# Autodesk Inventor assembly: PP
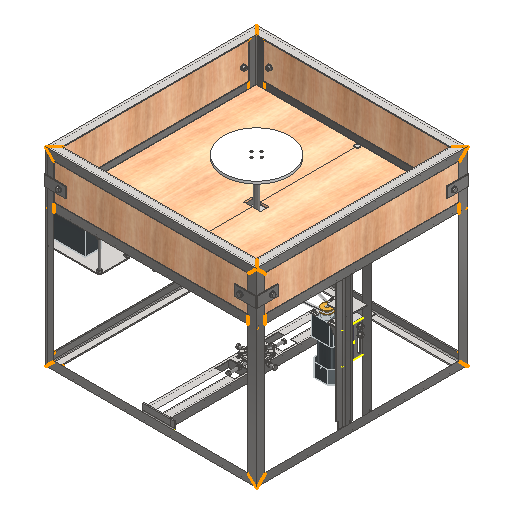
[picture p0: Inventor's stored thumbnail of the model, 512x512]
Saved by Autodesk Inventor 2025 (Build 290162000, 162)
## iProperties
Created: 2025-02-12
Part Number: PP
Document SubType Name: Weldment
Designer: teiko
Weld Material: Steel, Mild, Welded
Mass: 4.42779e+07 g
Surface Area: 1.45033e+06 cm^2
Volume: 5.65311e+06 cm^3
Density: 7.83248 g/cm^3
Author: teiko
## Documents named in this file (22)
- C:\Users\teiko\OneDrive\Documents\Inventor\Projectpotterpro\parts\PP.iam
- C:\Users\teiko\OneDrive\Documents\Inventor\Projectpotterpro\assembly\PP0101.iam
- C:\Users\teiko\OneDrive\Documents\Inventor\Projectpotterpro\parts\PP0306.iam
- C:\Users\teiko\OneDrive\Documents\Inventor\Content Center Files\R2025\en-US\ISO 7091\ISO 7091 - ST 12 - 100 HV.ipt
- C:\Users\teiko\OneDrive\Documents\Inventor\Content Center Files\R2025\en-US\ISO 4017(1)\ISO 4017 - M12 x 25 - ISO.ipt
- C:\Users\teiko\OneDrive\Documents\Inventor\Content Center Files\R2025\en-US\ISO 4032(2)\ISO 4032 - M12 - ISO.ipt
- C:\Users\teiko\OneDrive\Documents\Inventor\Projectpotterpro\parts\PP0501.ipt
- C:\Users\teiko\OneDrive\Documents\Inventor\Projectpotterpro\parts\PP0502.ipt
- C:\Users\teiko\OneDrive\Documents\Inventor\Projectpotterpro\parts\ISO 657-1 - L40x40x3-647.ipt
- C:\Users\teiko\OneDrive\Documents\Inventor\Projectpotterpro\parts\PP0411.iam
- C:\Users\teiko\OneDrive\Documents\Inventor\Projectpotterpro\parts\PP0412.ipt
- C:\Users\teiko\OneDrive\Documents\Inventor\Projectpotterpro\parts\PP0204.iam
- C:\Users\teiko\OneDrive\Documents\Inventor\Projectpotterpro\parts\6245K16_Pulley\6245K16_Pulley.ipt
- C:\Users\teiko\OneDrive\Documents\Inventor\Projectpotterpro\parts\PP0503.ipt
- C:\Users\teiko\OneDrive\Documents\Inventor\Content Center Files\R2025\en-US\ISO 4017(1)\ISO 4017 - M12 x 30 - ISO.ipt
- C:\Users\teiko\OneDrive\Documents\Inventor\Projectpotterpro\parts\PP0505.ipt
- C:\Users\teiko\OneDrive\Documents\Inventor\Projectpotterpro\parts\6245K541_Pulley\6245K541_Pulley.ipt
- C:\Users\teiko\OneDrive\Documents\Inventor\Projectpotterpro\parts\PP0504.ipt
- C:\Users\teiko\OneDrive\Documents\Inventor\Projectpotterpro\parts\PP\Design Accelerator\V-Belt transmission2.iam
- C:\Users\teiko\OneDrive\Documents\Inventor\Projectpotterpro\parts\PP0507.iam
- C:\Users\teiko\OneDrive\Documents\Inventor\Projectpotterpro\parts\PP0509.ipt
- C:\Users\teiko\OneDrive\Documents\Inventor\Projectpotterpro\parts\PP0510.ipt
## Components (79 placed, 21 different names)
1. PP0101:1 [sub-assembly] — Flush:1, Flush:2, Mate:1, Mate:5, Mate:6, Mate:7, Mate:9, Mate:10, Mate:11, Flush:10, Mate:31, Flush:18, Flush:19, Flush:22, Mate:51, Mate:73, Mate:74, Mate:81, Symmetry:2, Mate:92, Mate:93, Mate:106, Flush:97, Symmetry:3, Mate:107, Flush:98, Mate:109, Flush:100, Mate:115, Flush:104, Mate:125, Flush:108, Mate:130, Flush:109, Mate:131, Flush:111, Mate:132, Flush:114, Mate:133, Flush:116, Mate:134, Flush:118, Mate:135, Flush:120, Flush:122, Flush:123, Mate:154, Mate:155, Mate:163, Mate:164, Mate:165, Mate:170, Mate:172, Mate:178, Mate:180
2. ISO 7091 ST 12 - 100 HV:1 — Mate:5, Mate:6, Insert:1
3. ISO 4017 M12 x 25:1 — Insert:1, Mate:153
4. ISO 7091 ST 12 - 100 HV:2 — Mate:7, Insert:2
5. ISO 4032 M12:1 — Insert:2
6. ISO 7091 ST 12 - 100 HV:3 — Mate:9, Mate:10, Insert:3
7. ISO 4017 M12 x 25:2 — Insert:3, Mate:77, Mate:152
8. ISO 7091 ST 12 - 100 HV:4 — Mate:11, Mate:78
9. ISO 4032 M12:2 — Mate:77, Mate:78
10. PP0501:2 — Mate:92, Mate:93, Mate:114, Mate:119
11. PP0501:4 — Mate:107, Flush:98, Mate:108, Mate:124, Mate:129
12. PP0502:1 — Mate:31, Flush:18, Flush:19, Mate:52, Mate:53, Mate:83, Symmetry:3
13. PP0502:2 — Mate:51, Mate:52, Mate:53, Symmetry:2
14. ISO 657-1 - L40x40x3-647:1 — Mate:73, Mate:74, Mate:75, Flush:66, Symmetry:1
15. ISO 657-1 - L40x40x3-647:2 — Flush:66, Mate:81, Flush:67, Mate:82, Symmetry:1
16. PP0411:1 [sub-assembly] — Mate:82, Mate:83, Flush:68, Mate:84, Mate:96, Flush:124
17. PP0412:1 — Flush:69, Flush:70, Mate:85, Angle:1
18. ISO 4032 M12:3 — Mate:84, Mate:85, Angle:1
19. 6245K16_Pulley:1 — Mate:96, Flush:124, Flush:128
20. PP0503:1 — Mate:132, Flush:113, Flush:114, Flush:115, Mate:136, Mate:137, Mate:138
21. PP0503:2 — Mate:133, Flush:115, Flush:116, Flush:117, Mate:140, Mate:141, Mate:142
22. PP0503:3 — Mate:106, Flush:97, Mate:111, Mate:112, Mate:113, Flush:103, Flush:107
23. PP0503:4 — Mate:135, Flush:119, Flush:120, Mate:148, Mate:149, Mate:150
24. PP0503:7 — Mate:115, Flush:103, Flush:104, Mate:116, Mate:117, Mate:118, Flush:113, Flush:122
25. PP0503:8 — Mate:134, Flush:117, Flush:118, Mate:144, Mate:145, Mate:146
26. PP0503:9 — Mate:125, Flush:107, Flush:108, Mate:126, Mate:127, Mate:128
27. PP0503:10 — Mate:109, Flush:100, Mate:121, Mate:122, Mate:123, Flush:119, Flush:123
28. ISO 7091 ST 12 - 100 HV:5 — Mate:111, Mate:112, Insert:4
29. ISO 4017 M12 x 30:1 — Insert:4
30. ISO 7091 ST 12 - 100 HV:6 — Mate:113, Mate:114, Insert:5
31. ISO 4032 M12:4 — Insert:5
32. ISO 7091 ST 12 - 100 HV:7 — Mate:116, Mate:117, Insert:6
33. ISO 4017 M12 x 30:2 — Insert:6
34. ISO 7091 ST 12 - 100 HV:8 — Mate:118, Mate:119, Insert:7
35. ISO 4032 M12:5 — Insert:7
36. ISO 7091 ST 12 - 100 HV:9 — Mate:121, Mate:122, Insert:8
37. ISO 4017 M12 x 30:3 — Insert:8
38. ISO 7091 ST 12 - 100 HV:10 — Mate:123, Mate:124, Insert:9
39. ISO 4032 M12:6 — Insert:9
40. ISO 7091 ST 12 - 100 HV:11 — Mate:126, Mate:127, Insert:10
41. ISO 4017 M12 x 30:4 — Insert:10
42. ISO 7091 ST 12 - 100 HV:12 — Mate:128, Mate:129, Insert:11
43. ISO 4032 M12:7 — Insert:11
44. PP0505:1 — Mate:131, Flush:111, Flush:112, Mate:147, Mate:151
45. PP0505:2 — Mate:130, Flush:109, Flush:110, Mate:139, Mate:143
46. ISO 7091 ST 12 - 100 HV:13 — Mate:136, Mate:137, Insert:12
47. ISO 4017 M12 x 30:5 — Insert:12
48. ISO 7091 ST 12 - 100 HV:14 — Mate:138, Mate:139, Insert:13
49. ISO 4032 M12:8 — Insert:13
50. ISO 7091 ST 12 - 100 HV:15 — Mate:140, Mate:141, Insert:14
51. ISO 4017 M12 x 30:6 — Insert:14
52. ISO 7091 ST 12 - 100 HV:16 — Mate:142, Mate:143, Insert:15
53. ISO 4032 M12:9 — Insert:15
54. ISO 7091 ST 12 - 100 HV:17 — Mate:144, Mate:145, Insert:16
55. ISO 4017 M12 x 30:7 — Insert:16
56. ISO 7091 ST 12 - 100 HV:18 — Mate:146, Mate:147, Insert:17
57. ISO 4032 M12:10 — Insert:17
58. ISO 7091 ST 12 - 100 HV:19 — Mate:148, Mate:149, Insert:18
59. ISO 4017 M12 x 30:8 — Insert:18
60. ISO 7091 ST 12 - 100 HV:20 — Mate:150, Mate:151, Insert:19
61. ISO 4032 M12:11 — Insert:19
62. PP0306:1 [sub-assembly] — Mate:152, Mate:153, Mate:154, Flush:125, Flush:126
63. PP0306:2 [sub-assembly] — Flush:125, Flush:126, Mate:155, Mate:156, Flush:127
64. PP0204:1 [sub-assembly] — Mate:156, Flush:127, Mate:157, Mate:158, Mate:159, Mate:160, Mate:161
65. 6245K541_Pulley:1 — Mate:157, Flush:128, Mate:158
66. PP0504:1 — Mate:159, Mate:160, Mate:161
67. V-Belt transmission:1 [sub-assembly]
68. PP0507:1 [sub-assembly] — Mate:166, Mate:167, Mate:168, Flush:129
69. PP0509:1 — Mate:163, Mate:164, Mate:165, Insert:20, Insert:21, Insert:22, Insert:23, Mate:166, Mate:167, Mate:168, Flush:129, Mate:174, Mate:176
70. ISO 4032 M12:12 — Insert:20, Mate:169, Mate:175
71. ISO 4032 M12:13 — Insert:21, Mate:171, Mate:173
72. ISO 4032 M12:14 — Insert:22, Mate:177, Mate:179
73. ISO 4032 M12:15 — Insert:23
74. ISO 4032 M12:16 — Mate:169, Mate:170
75. ISO 4032 M12:17 — Mate:171, Mate:172
76. PP0510:1 — Mate:173, Mate:174
77. PP0510:2 — Mate:175, Mate:176
78. PP0510:3 — Mate:179, Mate:180
79. ISO 4032 M12:18 — Mate:177, Mate:178
## Relationships (162: Mate 96, Flush 39, Insert 23, Symmetry 3, Angle 1)
- Flush:1: PP0101:1
- Flush:2: PP0101:1
- Mate:1: PP0101:1
- Mate:5: PP0101:1 ↔ ISO 7091 ST 12 - 100 HV:1
- Mate:6: PP0101:1 ↔ ISO 7091 ST 12 - 100 HV:1
- Insert:1: ISO 7091 ST 12 - 100 HV:1 ↔ ISO 4017 M12 x 25:1
- Mate:7: PP0101:1 ↔ ISO 7091 ST 12 - 100 HV:2
- Insert:2: ISO 7091 ST 12 - 100 HV:2 ↔ ISO 4032 M12:1
- Mate:9: PP0101:1 ↔ ISO 7091 ST 12 - 100 HV:3
- Mate:10: PP0101:1 ↔ ISO 7091 ST 12 - 100 HV:3
- Insert:3: ISO 7091 ST 12 - 100 HV:3 ↔ ISO 4017 M12 x 25:2
- Mate:11: PP0101:1 ↔ ISO 7091 ST 12 - 100 HV:4
- Flush:10 (648.895 mm): PP0101:1
- Flush:12
- Mate:31: PP0101:1 ↔ PP0502:1
- Flush:18: PP0101:1 ↔ PP0502:1
- Flush:19: PP0101:1 ↔ PP0502:1
- Flush:22 (426.446 mm): PP0101:1
- Mate:51: PP0101:1 ↔ PP0502:2
- Mate:52: PP0502:1 ↔ PP0502:2
- Mate:53: PP0502:1 ↔ PP0502:2
- Mate:73: PP0101:1 ↔ ISO 657-1 - L40x40x3-647:1
- Mate:74 (-40 mm): PP0101:1 ↔ ISO 657-1 - L40x40x3-647:1
- Mate:75 (45 mm): ISO 657-1 - L40x40x3-647:1
- Mate:77: ISO 4017 M12 x 25:2 ↔ ISO 4032 M12:2
- Mate:78: ISO 7091 ST 12 - 100 HV:4 ↔ ISO 4032 M12:2
- Flush:66: ISO 657-1 - L40x40x3-647:1 ↔ ISO 657-1 - L40x40x3-647:2
- Mate:81: PP0101:1 ↔ ISO 657-1 - L40x40x3-647:2
- Flush:67 (-45 mm): ISO 657-1 - L40x40x3-647:2
- Mate:82: ISO 657-1 - L40x40x3-647:2 ↔ PP0411:1
- Symmetry:1: ISO 657-1 - L40x40x3-647:1 ↔ ISO 657-1 - L40x40x3-647:2
- Mate:83 (250 mm): PP0502:1 ↔ PP0411:1
- Flush:68 (60 mm): PP0411:1
- Flush:69: PP0412:1
- Flush:70: PP0412:1
- Mate:84: PP0411:1 ↔ ISO 4032 M12:3
- Mate:85: PP0412:1 ↔ ISO 4032 M12:3
- Angle:1 (0 deg): PP0412:1 ↔ ISO 4032 M12:3
- Symmetry:2: PP0101:1 ↔ PP0502:2
- Mate:92: PP0101:1 ↔ PP0501:2
- Mate:93: PP0101:1 ↔ PP0501:2
- Mate:96: PP0411:1 ↔ 6245K16_Pulley:1
- Mate:106: PP0101:1 ↔ PP0503:3
- Flush:97: PP0101:1 ↔ PP0503:3
- Symmetry:3: PP0101:1 ↔ PP0502:1
- Mate:107 (-3 mm): PP0101:1 ↔ PP0501:4
- Flush:98: PP0101:1 ↔ PP0501:4
- Mate:108: PP0501:4
- Mate:109: PP0101:1 ↔ PP0503:10
- Flush:100: PP0101:1 ↔ PP0503:10
- Mate:111: PP0503:3 ↔ ISO 7091 ST 12 - 100 HV:5
- Mate:112: PP0503:3 ↔ ISO 7091 ST 12 - 100 HV:5
- Insert:4: ISO 7091 ST 12 - 100 HV:5 ↔ ISO 4017 M12 x 30:1
- Mate:113: PP0503:3 ↔ ISO 7091 ST 12 - 100 HV:6
- Mate:114: PP0501:2 ↔ ISO 7091 ST 12 - 100 HV:6
- Insert:5: ISO 7091 ST 12 - 100 HV:6 ↔ ISO 4032 M12:4
- Mate:115: PP0101:1 ↔ PP0503:7
- Flush:103: PP0503:3 ↔ PP0503:7
- Flush:104: PP0101:1 ↔ PP0503:7
- Mate:116: PP0503:7 ↔ ISO 7091 ST 12 - 100 HV:7
- Mate:117: PP0503:7 ↔ ISO 7091 ST 12 - 100 HV:7
- Insert:6: ISO 7091 ST 12 - 100 HV:7 ↔ ISO 4017 M12 x 30:2
- Mate:118: PP0503:7 ↔ ISO 7091 ST 12 - 100 HV:8
- Mate:119: PP0501:2 ↔ ISO 7091 ST 12 - 100 HV:8
- Insert:7: ISO 7091 ST 12 - 100 HV:8 ↔ ISO 4032 M12:5
- Mate:121: PP0503:10 ↔ ISO 7091 ST 12 - 100 HV:9
- Mate:122: PP0503:10 ↔ ISO 7091 ST 12 - 100 HV:9
- Insert:8: ISO 7091 ST 12 - 100 HV:9 ↔ ISO 4017 M12 x 30:3
- Mate:123: PP0503:10 ↔ ISO 7091 ST 12 - 100 HV:10
- Mate:124: PP0501:4 ↔ ISO 7091 ST 12 - 100 HV:10
- Insert:9: ISO 7091 ST 12 - 100 HV:10 ↔ ISO 4032 M12:6
- Mate:125: PP0101:1 ↔ PP0503:9
- Flush:107: PP0503:3 ↔ PP0503:9
- Flush:108: PP0101:1 ↔ PP0503:9
- Mate:126: PP0503:9 ↔ ISO 7091 ST 12 - 100 HV:11
- Mate:127: PP0503:9 ↔ ISO 7091 ST 12 - 100 HV:11
- Insert:10: ISO 7091 ST 12 - 100 HV:11 ↔ ISO 4017 M12 x 30:4
- Mate:128: PP0503:9 ↔ ISO 7091 ST 12 - 100 HV:12
- Mate:129: PP0501:4 ↔ ISO 7091 ST 12 - 100 HV:12
- Insert:11: ISO 7091 ST 12 - 100 HV:12 ↔ ISO 4032 M12:7
- Mate:130 (-3 mm): PP0101:1 ↔ PP0505:2
- Flush:109: PP0101:1 ↔ PP0505:2
- Flush:110: PP0505:2
- Mate:131 (-3 mm): PP0101:1 ↔ PP0505:1
- Flush:111: PP0101:1 ↔ PP0505:1
- Flush:112: PP0505:1
- Mate:132: PP0101:1 ↔ PP0503:1
- Flush:113: PP0503:1 ↔ PP0503:7
- Flush:114: PP0101:1 ↔ PP0503:1
- Mate:133: PP0101:1 ↔ PP0503:2
- Flush:115: PP0503:1 ↔ PP0503:2
- Flush:116: PP0101:1 ↔ PP0503:2
- Mate:134: PP0101:1 ↔ PP0503:8
- Flush:117: PP0503:2 ↔ PP0503:8
- Flush:118: PP0101:1 ↔ PP0503:8
- Mate:135: PP0101:1 ↔ PP0503:4
- Flush:119: PP0503:4 ↔ PP0503:10
- Flush:120: PP0101:1 ↔ PP0503:4
- Mate:136: PP0503:1 ↔ ISO 7091 ST 12 - 100 HV:13
- Mate:137: PP0503:1 ↔ ISO 7091 ST 12 - 100 HV:13
- Insert:12: ISO 7091 ST 12 - 100 HV:13 ↔ ISO 4017 M12 x 30:5
- Mate:138: PP0503:1 ↔ ISO 7091 ST 12 - 100 HV:14
- Mate:139: PP0505:2 ↔ ISO 7091 ST 12 - 100 HV:14
- Insert:13: ISO 7091 ST 12 - 100 HV:14 ↔ ISO 4032 M12:8
- Mate:140: PP0503:2 ↔ ISO 7091 ST 12 - 100 HV:15
- Mate:141: PP0503:2 ↔ ISO 7091 ST 12 - 100 HV:15
- Insert:14: ISO 7091 ST 12 - 100 HV:15 ↔ ISO 4017 M12 x 30:6
- Mate:142: PP0503:2 ↔ ISO 7091 ST 12 - 100 HV:16
- Mate:143: PP0505:2 ↔ ISO 7091 ST 12 - 100 HV:16
- Insert:15: ISO 7091 ST 12 - 100 HV:16 ↔ ISO 4032 M12:9
- Mate:144: PP0503:8 ↔ ISO 7091 ST 12 - 100 HV:17
- Mate:145: PP0503:8 ↔ ISO 7091 ST 12 - 100 HV:17
- Insert:16: ISO 7091 ST 12 - 100 HV:17 ↔ ISO 4017 M12 x 30:7
- Mate:146: PP0503:8 ↔ ISO 7091 ST 12 - 100 HV:18
- Mate:147: PP0505:1 ↔ ISO 7091 ST 12 - 100 HV:18
- Insert:17: ISO 7091 ST 12 - 100 HV:18 ↔ ISO 4032 M12:10
- Mate:148: PP0503:4 ↔ ISO 7091 ST 12 - 100 HV:19
- Mate:149: PP0503:4 ↔ ISO 7091 ST 12 - 100 HV:19
- Insert:18: ISO 7091 ST 12 - 100 HV:19 ↔ ISO 4017 M12 x 30:8
- Mate:150: PP0503:4 ↔ ISO 7091 ST 12 - 100 HV:20
- Mate:151: PP0505:1 ↔ ISO 7091 ST 12 - 100 HV:20
- Insert:19: ISO 7091 ST 12 - 100 HV:20 ↔ ISO 4032 M12:11
- Flush:122 (112 mm): PP0101:1 ↔ PP0503:7
- Flush:123 (112 mm): PP0101:1 ↔ PP0503:10
- Flush:124: PP0411:1 ↔ 6245K16_Pulley:1
- Mate:152: ISO 4017 M12 x 25:2 ↔ PP0306:1
- Mate:153: ISO 4017 M12 x 25:1 ↔ PP0306:1
- Mate:154: PP0101:1 ↔ PP0306:1
- Flush:125: PP0306:1 ↔ PP0306:2
- Flush:126: PP0306:1 ↔ PP0306:2
- Mate:155: PP0101:1 ↔ PP0306:2
- Mate:156: PP0306:2 ↔ PP0204:1
- Flush:127: PP0306:2 ↔ PP0204:1
- Mate:157: PP0204:1 ↔ 6245K541_Pulley:1
- Flush:128: 6245K16_Pulley:1 ↔ 6245K541_Pulley:1
- Mate:158: PP0204:1 ↔ 6245K541_Pulley:1
- Mate:159: PP0204:1 ↔ PP0504:1
- Mate:160: PP0204:1 ↔ PP0504:1
- Mate:161: PP0204:1 ↔ PP0504:1
- Mate:163: PP0101:1 ↔ PP0509:1
- Mate:164: PP0101:1 ↔ PP0509:1
- Mate:165 (150 mm): PP0101:1 ↔ PP0509:1
- Insert:20: PP0509:1 ↔ ISO 4032 M12:12
- Insert:21: PP0509:1 ↔ ISO 4032 M12:13
- Insert:22: PP0509:1 ↔ ISO 4032 M12:14
- Insert:23: PP0509:1 ↔ ISO 4032 M12:15
- Mate:166: PP0507:1 ↔ PP0509:1
- Mate:167: PP0507:1 ↔ PP0509:1
- Mate:168 (3 mm): PP0507:1 ↔ PP0509:1
- Flush:129 (25 mm): PP0507:1 ↔ PP0509:1
- Mate:169: ISO 4032 M12:12 ↔ ISO 4032 M12:16
- Mate:170: PP0101:1 ↔ ISO 4032 M12:16
- Mate:171: ISO 4032 M12:13 ↔ ISO 4032 M12:17
- Mate:172: PP0101:1 ↔ ISO 4032 M12:17
- Mate:173: ISO 4032 M12:13 ↔ PP0510:1
- Mate:174: PP0509:1 ↔ PP0510:1
- Mate:175: ISO 4032 M12:12 ↔ PP0510:2
- Mate:176: PP0509:1 ↔ PP0510:2
- Mate:177: ISO 4032 M12:14 ↔ ISO 4032 M12:18
- Mate:178: PP0101:1 ↔ ISO 4032 M12:18
- Mate:179: ISO 4032 M12:14 ↔ PP0510:3
- Mate:180: PP0101:1 ↔ PP0510:3
